# Autodesk Inventor assembly: RFC522_PICO 1
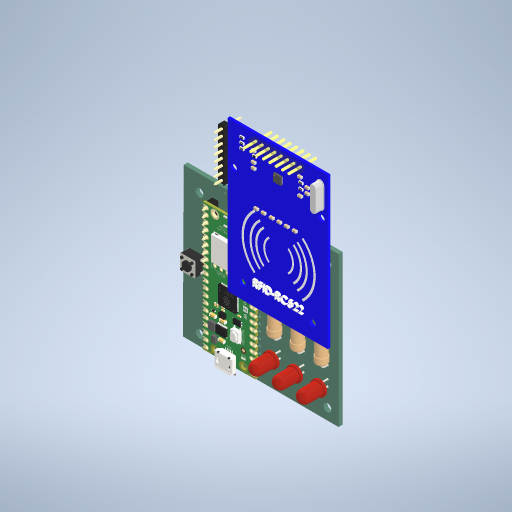
[picture p0: Inventor's stored thumbnail of the model, 512x512]
Saved by Autodesk Inventor 2024 (Build 280153000, 153)
## iProperties
Company: Kicad
Created: 2026-03-18
Part Number: RFC522_PICO 1
Description: KiCad electronic assembly
Document SubType Name: Assembly
Designer: volen
Authority: Unknown
Sending System: KiCad to STEP converter
Preprocessor: Open CASCADE STEP processor 7.8
Title: RFC522_PICO.step
Author: Pcbnew
## Documents named in this file (9)
- C:\Users\volen\Desktop\RFID reade_case\RFID_Board_plan\RFC522_PICO\RFC522_PICO.iam
- C:\Users\volen\Desktop\RFID reade_case\RFID_Board_plan\RFC522_PICO\R_Axial_DIN0414_L11.9mm_D4.5mm_P15.24mm_Horizontal.iam
- C:\Users\volen\Desktop\RFID reade_case\RFID_Board_plan\RFC522_PICO\Buzzer_12x9.5RM7.6.iam
- C:\Users\volen\Desktop\RFID reade_case\RFID_Board_plan\RFC522_PICO\LED_D5.0mm.iam
- C:\Users\volen\Desktop\RFID reade_case\RFID_Board_plan\RFC522_PICO\SW_PUSH_6mm.iam
- C:\Users\volen\Desktop\RFID reade_case\RFID_Board_plan\RFC522_PICO\_autosave-RFC522_PICO_PCB.ipt
- C:\Users\volen\Desktop\RFID reade_case\Raspberry Pi Pico 2W CAD Reference Model - 6962342\files\Pi_Pico_2W_CAD_Reference\Pi_Pico_2W_CAD_Reference.ipt
- C:\Users\volen\Desktop\RFID reade_case\rc522-rfid-module-1.snapshot.3\RFID.iam
- C:\Users\volen\Desktop\RFID reade_case\8-pin-header-reference-model-1.snapshot.1\Stiftleiste\Stiftleiste.iam
## Components (13 placed, 12 different names)
1. 2 [sub-assembly]
2. 4 [sub-assembly]
3. 6 [sub-assembly]
4. 7 [sub-assembly]
5. 9 [sub-assembly]
6. 10 [sub-assembly]
7. 11 [sub-assembly]
8. 12 [sub-assembly]
9. 13 — Mate:1, Mate:2, Mate:3, Flush:1, Mate:5
10. Pi_Pico_2W_CAD_Reference:1 — Mate:1, Mate:2, Mate:4
11. RFID:1 [sub-assembly]
12. Stiftleiste:1 [sub-assembly] — Mate:3, Flush:1, Mate:4
13. Stiftleiste:2 [sub-assembly] — Mate:5
## Relationships (6: Mate 5, Flush 1)
- Mate:1: 13 ↔ Pi_Pico_2W_CAD_Reference:1
- Mate:2: 13 ↔ Pi_Pico_2W_CAD_Reference:1
- Mate:3: 13 ↔ Stiftleiste:1
- Flush:1 (5.6 mm): 13 ↔ Stiftleiste:1
- Mate:4: Pi_Pico_2W_CAD_Reference:1 ↔ Stiftleiste:1
- Mate:5: 13 ↔ Stiftleiste:2
